# Autodesk Inventor assembly: MidSquareFull
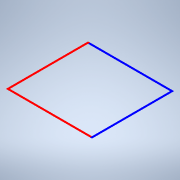
[picture p0: Inventor's stored thumbnail of the model, 180x180]
Saved by Autodesk Inventor 2021 (Build 250183000, 183)
## iProperties
Created: 2021-03-03
Part Number: MidSquareFull
Document SubType Name: Assembly
Designer: CMurray
Author: CMurray
## Documents named in this file (3)
- F:\PHRC CADD 2021\2021 Game Design Challenge\Full Field\Parts\Tape\MidSquareFull.iam
- F:\PHRC CADD 2021\2021 Game Design Challenge\Full Field\Parts\Tape\MidSquareRed1.ipt
- F:\PHRC CADD 2021\2021 Game Design Challenge\Full Field\Parts\Tape\MidSquareBlue1.ipt
## Components (4 placed, 2 different names)
1. MidSquareRed1:1 — Mate:1, Flush:1, Flush:2, Mate:3, Flush:5, Flush:6
2. MidSquareRed1:2 — Mate:1, Flush:1, Flush:2
3. MidSquareBlue1:1 — Flush:7, Mate:4, Flush:8
4. MidSquareBlue1:2 — Mate:3, Flush:5, Flush:6, Flush:7, Mate:4, Flush:8
## Relationships (9: Flush 6, Mate 3)
- Mate:1: MidSquareRed1:1 ↔ MidSquareRed1:2
- Flush:1: MidSquareRed1:1 ↔ MidSquareRed1:2
- Flush:2: MidSquareRed1:1 ↔ MidSquareRed1:2
- Mate:3: MidSquareRed1:1 ↔ MidSquareBlue1:2
- Flush:5: MidSquareRed1:1 ↔ MidSquareBlue1:2
- Flush:6: MidSquareRed1:1 ↔ MidSquareBlue1:2
- Flush:7: MidSquareBlue1:1 ↔ MidSquareBlue1:2
- Mate:4: MidSquareBlue1:1 ↔ MidSquareBlue1:2
- Flush:8: MidSquareBlue1:1 ↔ MidSquareBlue1:2
